# Autodesk Inventor assembly: Assembly2222
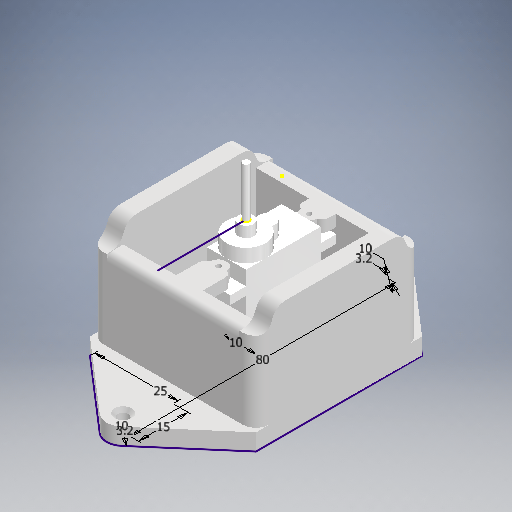
[picture p0: Inventor's stored thumbnail of the model, 512x512]
Saved by Autodesk Inventor 2025.3 (Build 293356000, 356)
## iProperties
Created: 2026-06-10
Part Number: Assembly2222
Document SubType Name: Assembly
Designer: user
Author: user
## Documents named in this file (3)
- C:\Ayman\Inventor Projects\Lifting Mechanism\Assembly2222.iam
- C:\Ayman\Inventor Projects\Lifting Mechanism\SERVO BASE HOUSING.Ayman.ipt
- C:\Ayman\Inventor Projects\Lifting Mechanism\SERVO.ipt
## Components (2 placed, 2 different names)
1. SERVO BASE HOUSING.Ayman:1 — Mate:1, Mate:2, Mate:3
2. SERVO:1 — Mate:1, Mate:2, Mate:3
## Relationships (3: Mate 3)
- Mate:1: SERVO BASE HOUSING.Ayman:1 ↔ SERVO:1
- Mate:2: SERVO BASE HOUSING.Ayman:1 ↔ SERVO:1
- Mate:3: SERVO BASE HOUSING.Ayman:1 ↔ SERVO:1
